# Autodesk Inventor assembly: Assembly1
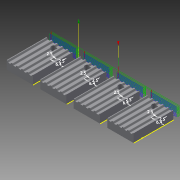
[picture p0: Inventor's stored thumbnail of the model, 180x180]
Saved by Autodesk Inventor 2015 SP1 (Build 190203100, 203)
## iProperties
Created: 2015-05-08
Part Number: Assembly1
Document SubType Name: Assembly
Designer: ubik
Author: ubik
## Documents named in this file (2)
- C:\Users\ubik\Dropbox\DueTech\cable test\Assembly1.iam
- C:\Users\ubik\Dropbox\DueTech\cable test\belt clamp.ipt
## Components (4 placed, 1 different names)
1. belt clamp:1 — Flush:1, Flush:2, Flush:3, Flush:4, Mate:1, Flush:6
2. belt clamp:2 — Flush:1, Flush:3, Mate:1, Mate:2
3. belt clamp:3 — Flush:2, Flush:4, Mate:2, Mate:3, Flush:5
4. belt clamp:4 — Mate:3, Flush:5, Flush:6
## Relationships (9: Flush 6, Mate 3)
- Flush:1: belt clamp:1 ↔ belt clamp:2
- Flush:2: belt clamp:1 ↔ belt clamp:3
- Flush:3: belt clamp:1 ↔ belt clamp:2
- Flush:4: belt clamp:1 ↔ belt clamp:3
- Mate:1 (3.5 mm): belt clamp:1 ↔ belt clamp:2
- Mate:2 (3.5 mm): belt clamp:2 ↔ belt clamp:3
- Mate:3 (3.5 mm): belt clamp:3 ↔ belt clamp:4
- Flush:5: belt clamp:3 ↔ belt clamp:4
- Flush:6: belt clamp:1 ↔ belt clamp:4
